# Autodesk Inventor assembly: Maquina de bolas
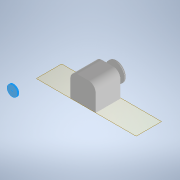
[picture p0: Inventor's stored thumbnail of the model, 180x180]
Saved by Autodesk Inventor 2020 (Build 240168000, 168)
## iProperties
Created: 2021-01-16
Part Number: Maquina de bolas
Document SubType Name: Assembly
Designer: pc-home
Author: pc-home
## Documents named in this file (4)
- D:\Bryan\ESPOL\2020- 2T\Diseño y Simulación de Máquinas\Proyecto2\proyecto2\Maquina de bolas.iam
- D:\Bryan\ESPOL\2020- 2T\Diseño y Simulación de Máquinas\Proyecto2\proyecto2\Motor DC\Pieza3.ipt
- D:\Bryan\ESPOL\2020- 2T\Diseño y Simulación de Máquinas\Inventor\Cadena1.ipt
- D:\Bryan\ESPOL\2020- 2T\Diseño y Simulación de Máquinas\Inventor\Cadena2.ipt
## Components (3 placed, 3 different names)
1. Pieza3:1 — Insertar:1
2. Cadena1:1 — Insertar:1
3. Cadena2:1
## Relationships (1: Insert 1)
- Insertar:1: Pieza3:1 ↔ Cadena1:1
